# Autodesk Inventor assembly: arm_half_mirrored
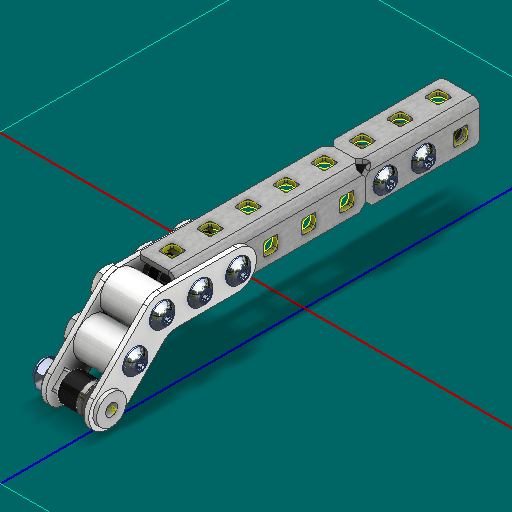
[picture p0: Inventor's stored thumbnail of the model, 512x512]
Saved by Autodesk Inventor 2025 (Build 290162000, 162)
## iProperties
Created: 2024-08-18
Part Number: arm_half_mirrored
Document SubType Name: Assembly
Designer: averey
Author: averey
## Documents named in this file (5)
- C:\Users\avere\vex_robotics_high_stakes\hardware\cad\ATLAS\intake\first_stage\arm\arm_half_mirrored\arm_half_mirrored.iam
- C:\Users\avere\vex_robotics_high_stakes\hardware\cad\ATLAS\intake\first_stage\arm\arm_half_mirrored\Alu Angle 1x1x8_mirrored.ipt
- C:\Users\avere\vex_robotics_high_stakes\hardware\cad\VEX-CAD-Inventor\Structure\Angle\Aluminum 1x1\Alu Angle 1x1x5.ipt
- C:\Users\avere\vex_robotics_high_stakes\hardware\cad\_quick_assemblies\bearing_flat_w_hardware_offset.iam
- C:\Users\avere\vex_robotics_high_stakes\hardware\cad\ATLAS\intake\first_stage\arm\gusset_mirrored\gusset_mirrored.iam
## Components (4 placed, 4 different names)
1. Alu Angle 1x1x8_mirrored:1 — Angle:2, Angle:1, Mate:2, Insert:8, Mate:7, Insert:9, Mate:8
2. Alu Angle 1x1x5:1
3. bearing_flat_w_hardware_offset:1 [sub-assembly] — Insert:8, Mate:7
4. gusset_mirrored:1 [sub-assembly] — Insert:9, Mate:8
## Relationships (7: Mate 3, Angle 2, Insert 2)
- Angle:2 (90 deg): Alu Angle 1x1x8_mirrored:1
- Angle:1 (0 deg): Alu Angle 1x1x8_mirrored:1
- Mate:2: Alu Angle 1x1x8_mirrored:1
- Insert:8: Alu Angle 1x1x8_mirrored:1 ↔ bearing_flat_w_hardware_offset:1
- Mate:7: Alu Angle 1x1x8_mirrored:1 ↔ bearing_flat_w_hardware_offset:1
- Insert:9: Alu Angle 1x1x8_mirrored:1 ↔ gusset_mirrored:1
- Mate:8: Alu Angle 1x1x8_mirrored:1 ↔ gusset_mirrored:1
